# Autodesk Inventor assembly: StepperMotor_Nema24
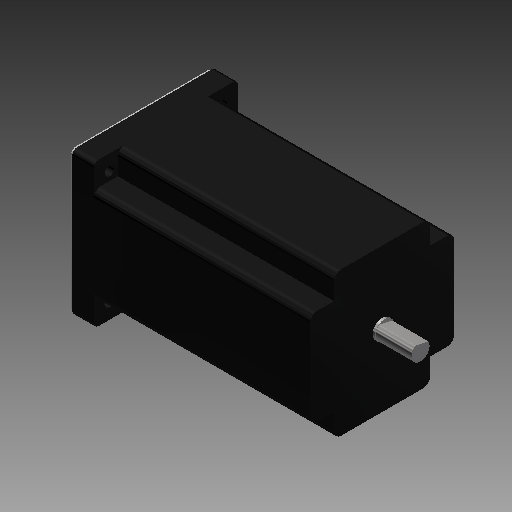
[picture p0: Inventor's stored thumbnail of the model, 512x512]
Saved by Autodesk Inventor 2017 SP1 (Build 210196100, 196)
## iProperties
Created: 2017-08-05
Part Number: StepperMotor_Nema24
Document SubType Name: Assembly
Designer: Zach
Author: Zach
## Documents named in this file (5)
- C:\Users\Zach\Documents\GitHub\cr-laundry-robot\lib\Stepper Motor - NEMA 24\StepperMotor_Nema24.iam
- C:\Users\Zach\Documents\GitHub\cr-laundry-robot\lib\Stepper Motor - NEMA 24\Part1.ipt
- C:\Users\Zach\Documents\GitHub\cr-laundry-robot\lib\Stepper Motor - NEMA 24\Part2.ipt
- C:\Users\Zach\Documents\GitHub\cr-laundry-robot\lib\Stepper Motor - NEMA 24\Part3.ipt
- C:\Users\Zach\Documents\GitHub\cr-laundry-robot\lib\Stepper Motor - NEMA 24\Part4.ipt
## Components (4 placed, 4 different names)
1. Part1:1 — Mate:1, Mate:3, Mate:5, Mate:6, Mate:7, Mate:8
2. Part2:1 — Mate:1, Mate:4, Flush:1
3. Part3:1 — Mate:3, Mate:4, Mate:5, Mate:6
4. Part4:1 — Mate:7, Mate:8, Flush:1
## Relationships (8: Mate 7, Flush 1)
- Mate:1: Part1:1 ↔ Part2:1
- Mate:3: Part1:1 ↔ Part3:1
- Mate:4: Part2:1 ↔ Part3:1
- Mate:5: Part1:1 ↔ Part3:1
- Mate:6: Part1:1 ↔ Part3:1
- Mate:7: Part1:1 ↔ Part4:1
- Mate:8: Part1:1 ↔ Part4:1
- Flush:1: Part2:1 ↔ Part4:1
